# Autodesk Inventor assembly: ControllerAssembly
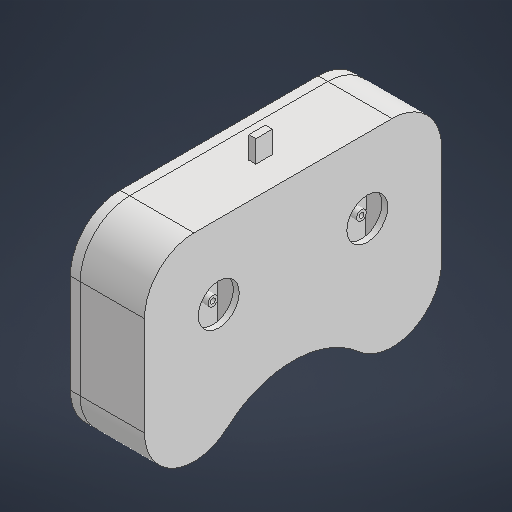
[picture p0: Inventor's stored thumbnail of the model, 512x512]
Saved by Autodesk Inventor 2026.1 (Build 301233000, 233)
## iProperties
Created: 2026-07-06
Part Number: ControllerAssembly
Document SubType Name: Assembly
Designer: Kasi Pusuluri
Author: Kasi Pusuluri
## Documents named in this file (8)
- C:\Users\Kasi Pusuluri\Documents\Outpost 2026\Controller\ControllerAssembly.iam
- C:\Users\Kasi Pusuluri\Documents\Outpost 2026\Controller\ControllerTop.ipt
- C:\Users\Kasi Pusuluri\Documents\Outpost 2026\Controller\ControllerBottom.ipt
- C:\Users\Kasi Pusuluri\Documents\Outpost 2026\BumperCarV2\PCB2.ipt
- C:\Users\Kasi Pusuluri\Documents\Outpost 2026\Controller\BatteryHolder.ipt
- C:\Users\Kasi Pusuluri\Documents\Outpost 2026\BumperCarV2\NRF24L01+.ipt
- C:\Users\Kasi Pusuluri\Documents\Outpost 2026\Controller\SlideSwitch.ipt
- C:\Users\Kasi Pusuluri\Documents\Outpost 2026\Controller\VoltageRegulator.ipt
## Components (7 placed, 7 different names)
1. ControllerTop:1 — Rigid:1, Mate:3, Mate:4, Mate:5, Mate:6, Mate:7, Mate:8
2. ControllerBottom:1 — Mate:7, Mate:8
3. PCB2:1
4. BatteryHolder:1 — Rigid:1
5. NRF24L01+:1
6. SlideSwitch:1 — Mate:3, Mate:4, Mate:5
7. VoltageRegulator:1 — Mate:6
## Relationships (7: Mate 6, WeldJoint 1)
- Rigid:1 [WeldJoint]: ControllerTop:1 ↔ BatteryHolder:1
- Mate:3: ControllerTop:1 ↔ SlideSwitch:1
- Mate:4: ControllerTop:1 ↔ SlideSwitch:1
- Mate:5: ControllerTop:1 ↔ SlideSwitch:1
- Mate:6: ControllerTop:1 ↔ VoltageRegulator:1
- Mate:7: ControllerTop:1 ↔ ControllerBottom:1
- Mate:8: ControllerTop:1 ↔ ControllerBottom:1
